# Autodesk Inventor assembly: frame
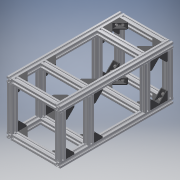
[picture p0: Inventor's stored thumbnail of the model, 180x180]
Saved by Autodesk Inventor 2016 (Build 200138000, 138)
## iProperties
Created: 2016-07-21
Part Number: frame
Document SubType Name: Assembly
Designer: Jonathan
Author: Jonathan
## Documents named in this file (4)
- C:\Users\Jonathan\Desktop\Models\Four Paddle Detector\frame\frame.iam
- C:\Users\Jonathan\Desktop\Models\Four Paddle Detector\frame\shapes\15x15.iam
- C:\Users\Jonathan\Desktop\Models\Four Paddle Detector\frame\extrusions\40 cm extrusion.ipt
- C:\Users\Jonathan\Desktop\Models\Four Paddle Detector\frameSpecifications.xlsx
## Components (8 placed, 2 different names)
1. 15x15:1 [sub-assembly] — Mate:1, Mate:2, Flush:1, Mate:3, Mate:4, Flush:2, Mate:5, Mate:6, Flush:3, Mate:7, Mate:8, Flush:4, Flush:6
2. 40 cm extrusion:1 — Mate:3, Mate:4, Flush:2
3. 40 cm extrusion:2 — Mate:1, Mate:2, Flush:1
4. 40 cm extrusion:3 — Mate:7, Mate:8, Flush:4, Mate:9, Mate:10, Flush:5, Mate:11, Mate:12, Mate:13, Mate:14
5. 40 cm extrusion:4 — Mate:5, Mate:6, Flush:3
6. 15x15:2 [sub-assembly] — Mate:9, Mate:10, Flush:5
7. 15x15:3 [sub-assembly] — Mate:12, Mate:13, Flush:7
8. 15x15:4 [sub-assembly] — Mate:11, Mate:14, Flush:6, Flush:7
## Relationships (21: Mate 14, Flush 7)
- Mate:1: 15x15:1 ↔ 40 cm extrusion:2
- Mate:2: 15x15:1 ↔ 40 cm extrusion:2
- Flush:1: 15x15:1 ↔ 40 cm extrusion:2
- Mate:3: 15x15:1 ↔ 40 cm extrusion:1
- Mate:4: 15x15:1 ↔ 40 cm extrusion:1
- Flush:2: 15x15:1 ↔ 40 cm extrusion:1
- Mate:5: 15x15:1 ↔ 40 cm extrusion:4
- Mate:6: 15x15:1 ↔ 40 cm extrusion:4
- Flush:3: 15x15:1 ↔ 40 cm extrusion:4
- Mate:7: 15x15:1 ↔ 40 cm extrusion:3
- Mate:8: 15x15:1 ↔ 40 cm extrusion:3
- Flush:4: 15x15:1 ↔ 40 cm extrusion:3
- Mate:9: 40 cm extrusion:3 ↔ 15x15:2
- Mate:10: 40 cm extrusion:3 ↔ 15x15:2
- Flush:5: 40 cm extrusion:3 ↔ 15x15:2
- Mate:11: 40 cm extrusion:3 ↔ 15x15:4
- Mate:12: 40 cm extrusion:3 ↔ 15x15:3
- Mate:13: 40 cm extrusion:3 ↔ 15x15:3
- Mate:14: 40 cm extrusion:3 ↔ 15x15:4
- Flush:6 (100 mm): 15x15:1 ↔ 15x15:4
- Flush:7 (-200 mm): 15x15:3 ↔ 15x15:4
## Named parameters: height = 400 mm, width = 150 mm, topSeparation = 100 mm, botSeparation = 200 mm, panelChamfer = 75 mm
